# Autodesk Inventor assembly: 試組
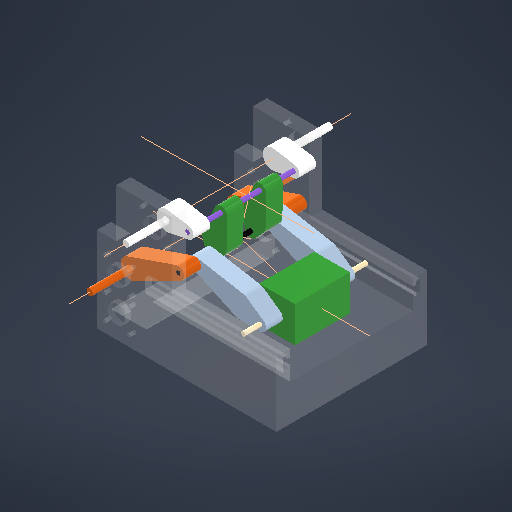
[picture p0: Inventor's stored thumbnail of the model, 512x512]
Saved by Autodesk Inventor 2025.3 (Build 293356030, 356C)
## iProperties
Created: 2025-08-27
Part Number: 試組
Document SubType Name: Assembly
Designer: 陳泓任
Author: 陳泓任
## Documents named in this file (8)
- C:\Users\Ou918\Downloads\AI-optimization\reference\model\試組.iam
- C:\Users\Ou918\Downloads\AI-optimization\reference\model\Type 1A R1前充座.ipt
- C:\Users\Ou918\Downloads\AI-optimization\reference\model\Type 1A R2延伸曲柄.ipt
- C:\Users\Ou918\Downloads\AI-optimization\reference\model\Type 1A R3延伸連接桿.ipt
- C:\Users\Ou918\Downloads\AI-optimization\reference\model\Type 1A R4主滑台曲柄.ipt
- C:\Users\Ou918\Downloads\AI-optimization\reference\model\Type 1A R5主滑台連接桿.ipt
- C:\Users\Ou918\Downloads\AI-optimization\reference\model\Type 1A R6主滑台_modified.ipt
- C:\Users\Ou918\Downloads\AI-optimization\reference\model\Type 1A 連接軸 1.ipt
## Components (9 placed, 7 different names)
1. Type 1A R1前充座:1 — J12, 旋轉:3, 滑塊:1
2. Type 1A R2延伸曲柄:1 — J12, 角度:1, 剛性:1, J23
3. Type 1A R3延伸連接桿:1 — J23, 貼合:R3-R5, 同軸R3
4. Type 1A R4主滑台曲柄:1 — 旋轉:3, 剛性:2, J45
5. Type 1A R5主滑台連接桿:1 — J45, 剛性:3, 貼合:R3-R5
6. Type 1A R6主滑台_modified:1 — 滑塊:1, 貼合:3
7. Type 1A 連接軸 1:1 — 剛性:1
8. Type 1A 連接軸 1:2 — 剛性:2, 同軸R3
9. Type 1A 連接軸 1:3 — 剛性:3, 貼合:3
## Relationships (12: RevoluteJoint 3, WeldJoint 3, Mate 3, Angle 1, CylindricalJoint 1, TranslationJoint 1)
- J12 [RevoluteJoint]: Type 1A R1前充座:1 ↔ Type 1A R2延伸曲柄:1
- 角度:1 [Angle] (89 deg): Type 1A R2延伸曲柄:1
- 剛性:1 [WeldJoint]: Type 1A R2延伸曲柄:1 ↔ Type 1A 連接軸 1:1
- J23 [CylindricalJoint]: Type 1A R2延伸曲柄:1 ↔ Type 1A R3延伸連接桿:1
- 旋轉:3 [RevoluteJoint]: Type 1A R1前充座:1 ↔ Type 1A R4主滑台曲柄:1
- 剛性:2 [WeldJoint]: Type 1A R4主滑台曲柄:1 ↔ Type 1A 連接軸 1:2
- J45 [RevoluteJoint]: Type 1A R4主滑台曲柄:1 ↔ Type 1A R5主滑台連接桿:1
- 剛性:3 [WeldJoint] (-103 mm): Type 1A R5主滑台連接桿:1 ↔ Type 1A 連接軸 1:3
- 貼合:R3-R5 [Mate]: Type 1A R3延伸連接桿:1 ↔ Type 1A R5主滑台連接桿:1
- 同軸R3 [Mate]: Type 1A R3延伸連接桿:1 ↔ Type 1A 連接軸 1:2
- 滑塊:1 [TranslationJoint]: Type 1A R1前充座:1 ↔ Type 1A R6主滑台_modified:1
- 貼合:3 [Mate]: Type 1A R6主滑台_modified:1 ↔ Type 1A 連接軸 1:3
